# Autodesk Inventor assembly: BottomHopperAssembly
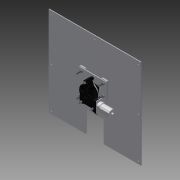
[picture p0: Inventor's stored thumbnail of the model, 180x180]
Saved by Autodesk Inventor 2013 (Build 170138000, 138)
## iProperties
Created: 2013-07-16
Part Number: BottomHopperAssembly
Document SubType Name: Assembly
Designer: orange
Author: orange
## Documents named in this file (5)
- H:\FRC_Projects\Cad\Inventor_Projects\Shooter_No_Welding\Hopper\BottomHopperAssembly.iam
- H:\FRC_Projects\Cad\Inventor_Projects\Shooter_No_Welding\Hopper\WindowMotorMounting.iam
- H:\FRC_Projects\Cad\Inventor_Projects\Shooter_No_Welding\Library\ANSI B18.6.3 - 1_4-20 UNC - 1.5(31).ipt
- H:\FRC_Projects\Cad\Inventor_Projects\Shooter_No_Welding\Library\AS 2465 - 1_4  UNC(1).ipt
- H:\FRC_Projects\Cad\Inventor_Projects\Shooter_No_Welding\Hopper\New BottomHopper Plate.ipt
## Components (10 placed, 4 different names)
1. WindowMotorMounting:1 [sub-assembly] — Mate:17, Mate:19, Mate:22, Mate:23, Mate:24, Mate:25, Mate:26, Mate:27, Mate:28, Mate:29, Mate:30, Mate:31, Mate:32
2. Large Hex Head Machine Screw - Inch 1/4-20 UNC - 1.5:1 — Mate:20, Mate:30, Mate:33
3. Large Hex Head Machine Screw - Inch 1/4-20 UNC - 1.5:2 — Mate:21, Mate:28, Mate:35
4. Large Hex Head Machine Screw - Inch 1/4-20 UNC - 1.5:3 — Mate:18, Mate:29, Mate:34
5. Large Hex Head Machine Screw - Inch 1/4-20 UNC - 1.5:4 — Mate:16, Mate:31, Mate:36
6. AS 2465 - Inch 1/4  UNC:1 — Mate:16, Mate:17
7. AS 2465 - Inch 1/4  UNC:2 — Mate:20, Mate:23
8. AS 2465 - Inch 1/4  UNC:3 — Mate:21, Mate:22
9. AS 2465 - Inch 1/4  UNC:4 — Mate:18, Mate:19
10. New BottomHopper Plate:1 — Mate:24, Mate:25, Mate:26, Mate:27, Mate:32, Mate:33, Mate:34, Mate:35, Mate:36
## Relationships (21: Mate 21)
- Mate:16: Large Hex Head Machine Screw - Inch 1/4-20 UNC - 1.5:4 ↔ AS 2465 - Inch 1/4  UNC:1
- Mate:17: WindowMotorMounting:1 ↔ AS 2465 - Inch 1/4  UNC:1
- Mate:18: Large Hex Head Machine Screw - Inch 1/4-20 UNC - 1.5:3 ↔ AS 2465 - Inch 1/4  UNC:4
- Mate:19: WindowMotorMounting:1 ↔ AS 2465 - Inch 1/4  UNC:4
- Mate:20: Large Hex Head Machine Screw - Inch 1/4-20 UNC - 1.5:1 ↔ AS 2465 - Inch 1/4  UNC:2
- Mate:21: Large Hex Head Machine Screw - Inch 1/4-20 UNC - 1.5:2 ↔ AS 2465 - Inch 1/4  UNC:3
- Mate:22: WindowMotorMounting:1 ↔ AS 2465 - Inch 1/4  UNC:3
- Mate:23: WindowMotorMounting:1 ↔ AS 2465 - Inch 1/4  UNC:2
- Mate:24: WindowMotorMounting:1 ↔ New BottomHopper Plate:1
- Mate:25: WindowMotorMounting:1 ↔ New BottomHopper Plate:1
- Mate:26: WindowMotorMounting:1 ↔ New BottomHopper Plate:1
- Mate:27: WindowMotorMounting:1 ↔ New BottomHopper Plate:1
- Mate:28: WindowMotorMounting:1 ↔ Large Hex Head Machine Screw - Inch 1/4-20 UNC - 1.5:2
- Mate:29: WindowMotorMounting:1 ↔ Large Hex Head Machine Screw - Inch 1/4-20 UNC - 1.5:3
- Mate:30: WindowMotorMounting:1 ↔ Large Hex Head Machine Screw - Inch 1/4-20 UNC - 1.5:1
- Mate:31: WindowMotorMounting:1 ↔ Large Hex Head Machine Screw - Inch 1/4-20 UNC - 1.5:4
- Mate:32: WindowMotorMounting:1 ↔ New BottomHopper Plate:1
- Mate:33: Large Hex Head Machine Screw - Inch 1/4-20 UNC - 1.5:1 ↔ New BottomHopper Plate:1
- Mate:34: Large Hex Head Machine Screw - Inch 1/4-20 UNC - 1.5:3 ↔ New BottomHopper Plate:1
- Mate:35: Large Hex Head Machine Screw - Inch 1/4-20 UNC - 1.5:2 ↔ New BottomHopper Plate:1
- Mate:36: Large Hex Head Machine Screw - Inch 1/4-20 UNC - 1.5:4 ↔ New BottomHopper Plate:1
